# Autodesk Inventor assembly: Etapa3
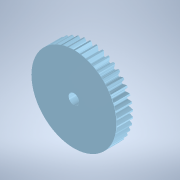
[picture p0: Inventor's stored thumbnail of the model, 180x180]
Saved by Autodesk Inventor 2022 (Build 260153000, 153)
## iProperties
Created: 2022-02-26
Part Number: Etapa3
Document SubType Name: Assembly
Designer: hurta
Author: hurta
## Documents named in this file (3)
- C:\Users\hurta\Documents\Universidad\NovenoSemestre\Diseno e Innovacion en Ingenieria\PoleaFaja\Etapa3.iam
- C:\Users\hurta\Documents\Universidad\NovenoSemestre\Diseno e Innovacion en Ingenieria\Engranes\Engrane42Dientes.ipt
- C:\Users\hurta\Documents\Universidad\NovenoSemestre\Diseno e Innovacion en Ingenieria\Engranes\Engrane14Dientes.ipt
## Components (2 placed, 2 different names)
1. Engrane42Dientes:1 — Mate:1, Mate:2
2. Engrane14Dientes:1 — Mate:1, Mate:2
## Relationships (2: Mate 2)
- Mate:1: Engrane42Dientes:1 ↔ Engrane14Dientes:1
- Mate:2: Engrane42Dientes:1 ↔ Engrane14Dientes:1
